# Autodesk Inventor assembly: Electrronic Enclosure
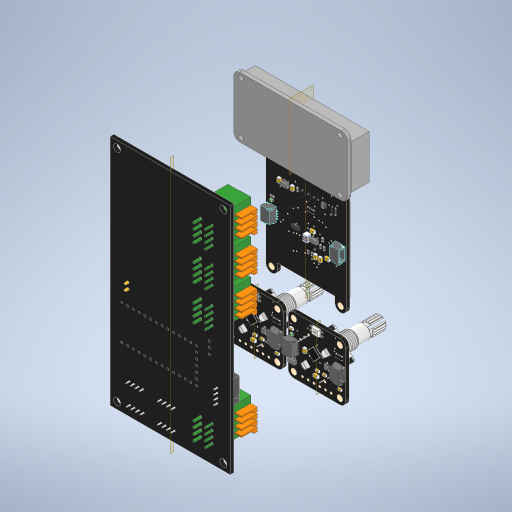
[picture p0: Inventor's stored thumbnail of the model, 512x512]
Saved by Autodesk Inventor 2023 (Build 270158000, 158)
## iProperties
Created: 2021-02-17
Part Number: Electrronic Enclosure
Document SubType Name: Assembly
Designer: jeffb
Sending System: Autodesk Translation Framework v9.7.0.1280
Preprocessor: ST-DEVELOPER v18.1
Title: /Users/emac5k/Dropbox/Adafruit/3D/Adafruit_CAD_Parts/4741 OLED 1.5in/Adafruit Grayscale 1.5-inch 128x128 OLED v2.step
## Documents named in this file (5)
- F:\OneDrive\Documents\Inventor\ELS\Electrronic Enclosure.iam
- F:\OneDrive\Documents\Inventor\ELS\1.5 inch oled\PCB Component.iam
- F:\OneDrive\Documents\Inventor\ELS\Encoder\4991 QT Rotary Encoder.iam
- F:\OneDrive\Documents\Inventor\ELS\878 7-segment display backpack.ipt
- F:\OneDrive\Documents\Inventor\ELS\main board\ELS Main Board.iam
## Components (5 placed, 4 different names)
1. PCB Component:1 [sub-assembly] — Angle:1, Angle:2, Angle:3, Angle:4, Flush:1, Angle:5, Angle:6, Mate:2, Mate:3, Mate:4, Mate:5
2. 4991 QT Rotary Encoder:1 [sub-assembly] — Angle:1, Angle:4, Mate:4, Flush:2, Flush:5, Flush:7
3. 4991 QT Rotary Encoder:2 [sub-assembly] — Angle:2, Angle:3, Flush:2, Flush:4, Flush:5, Flush:6
4. 878 7-segment display backpack:1 — Flush:1, Mate:1, Mate:2, Mate:3, Flush:3
5. ELS Main Board:1 [sub-assembly] — Angle:5, Angle:6, Mate:1, Flush:3, Flush:4, Flush:6, Flush:7, Mate:5
## Relationships (18: Flush 7, Angle 6, Mate 5)
- Angle:1 (0 deg): PCB Component:1 ↔ 4991 QT Rotary Encoder:1
- Angle:2 (0 deg): PCB Component:1 ↔ 4991 QT Rotary Encoder:2
- Angle:3 (0 deg): PCB Component:1 ↔ 4991 QT Rotary Encoder:2
- Angle:4 (0 deg): PCB Component:1 ↔ 4991 QT Rotary Encoder:1
- Flush:1: PCB Component:1 ↔ 878 7-segment display backpack:1
- Angle:5 (0 deg): PCB Component:1 ↔ ELS Main Board:1
- Angle:6 (0 deg): PCB Component:1 ↔ ELS Main Board:1
- Mate:1 (38.1 mm): 878 7-segment display backpack:1 ↔ ELS Main Board:1
- Mate:2 (3 mm): PCB Component:1 ↔ 878 7-segment display backpack:1
- Mate:3: PCB Component:1 ↔ 878 7-segment display backpack:1
- Mate:4 (1 mm): PCB Component:1 ↔ 4991 QT Rotary Encoder:1
- Flush:2: 4991 QT Rotary Encoder:1 ↔ 4991 QT Rotary Encoder:2
- Flush:3: 878 7-segment display backpack:1 ↔ ELS Main Board:1
- Flush:4: 4991 QT Rotary Encoder:2 ↔ ELS Main Board:1
- Flush:5: 4991 QT Rotary Encoder:1 ↔ 4991 QT Rotary Encoder:2
- Flush:6: 4991 QT Rotary Encoder:2 ↔ ELS Main Board:1
- Flush:7: 4991 QT Rotary Encoder:1 ↔ ELS Main Board:1
- Mate:5: PCB Component:1 ↔ ELS Main Board:1
